# Autodesk Inventor assembly: hotend
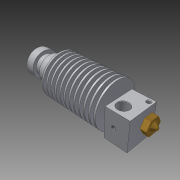
[picture p0: Inventor's stored thumbnail of the model, 180x180]
Saved by Autodesk Inventor 2014 (Build 180170000, 170)
## iProperties
Created: 2014-03-25
Part Number: hotend
Document SubType Name: Assembly
Designer: buben
Mass: 36.4823 g
Surface Area: 193.146 cm^2
Volume: 13.0647 cm^3
Density: 2.79244 g/cm^3
Author: buben
## Documents named in this file (6)
- C:\Users\buben\Documents\GitHub\bacon\inventor files\utils\ds_hotend\hotend.iam
- C:\Users\buben\Documents\GitHub\bacon\inventor files\utils\ds_hotend\hotend_mount.ipt
- C:\Users\buben\Documents\GitHub\bacon\inventor files\utils\ds_hotend\cooling_element.ipt
- C:\Users\buben\Documents\GitHub\bacon\inventor files\utils\ds_hotend\cooling_spacer.ipt
- C:\Users\buben\Documents\GitHub\bacon\inventor files\utils\ds_hotend\heatblock.ipt
- C:\Users\buben\Documents\GitHub\bacon\inventor files\utils\ds_hotend\nozzle.ipt
## Components (26 placed, 5 different names)
1. hotend_mount:1 — Mate:3, Mate:4, Mate:5, Mate:8, Mate:9, Mate:12, Mate:13
2. cooling_element:12 — Mate:6, Mate:7
3. heatblock:1 — Mate:8, Mate:9, Mate:10, Mate:11, Angle:1, Angle:2
4. nozzle:1 — Mate:10, Mate:11, Angle:1
5. cooling_spacer:1 — Mate:1, Mate:2, Mate:4
6. cooling_element:1 — Mate:1, Mate:2, Mate:3
7. cooling_spacer:2
8. cooling_element:2
9. cooling_spacer:3
10. cooling_element:3
11. cooling_spacer:4
12. cooling_element:4
13. cooling_spacer:5
14. cooling_element:5
15. cooling_spacer:6
16. cooling_element:6
17. cooling_spacer:7
18. cooling_element:7
19. cooling_spacer:8
20. cooling_element:8
21. cooling_spacer:9
22. cooling_element:9
23. cooling_spacer:10
24. cooling_element:10
25. cooling_spacer:11 — Mate:6
26. cooling_element:11
## Component patterns: (11 elements, first: cooling_spacer:1 + cooling_element:1)
## Relationships (15: Mate 13, Angle 2)
- Mate:1: cooling_spacer:1 ↔ cooling_element:1
- Mate:2: cooling_spacer:1 ↔ cooling_element:1
- Mate:3: hotend_mount:1 ↔ cooling_element:1
- Mate:4: hotend_mount:1 ↔ cooling_spacer:1
- Mate:5: hotend_mount:1
- Mate:6: cooling_element:12 ↔ cooling_spacer:11
- Mate:7: cooling_element:12
- Mate:8: hotend_mount:1 ↔ heatblock:1
- Mate:9: hotend_mount:1 ↔ heatblock:1
- Mate:10: heatblock:1 ↔ nozzle:1
- Mate:11: heatblock:1 ↔ nozzle:1
- Angle:1 (0 deg): heatblock:1 ↔ nozzle:1
- Mate:12: hotend_mount:1
- Mate:13: hotend_mount:1
- Angle:2 (180 deg): heatblock:1
